# Autodesk Inventor assembly: Motorkühlung
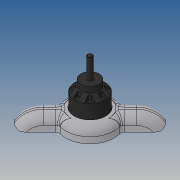
[picture p0: Inventor's stored thumbnail of the model, 180x180]
Saved by Autodesk Inventor 2019.4 (Build 234330000, 330)
## iProperties
Part Number: Motorkühlung
Document SubType Name: Assembly
Designer: Admin
Mass: 135.524 g
Surface Area: 242.561 cm^2
Volume: 41.9038 cm^3
Density: 3.23417 g/cm^3
Author: Admin
Revision: -
VAULT_Status: in Bearbeitung
Gewicht: 0,136 kg
InventorVersion: 2019.4
## Documents named in this file (4)
- C:\Users\tonn\Documents\GitHub\CAD_Elements\CAD\Hektor\Motorkühlung.iam
- Norm.iam
- C:\Users\tonn\Documents\GitHub\CAD_Elements\CAD\Motor\CobraCP2814-1050kv.ipt
- C:\Users\tonn\Documents\GitHub\CAD_Elements\CAD\Hektor\Motorkühlung.ipt
## Components (2 placed, 2 different names)
1. COBRACP2814-1050KV_COBRACP2814-1050KV--IPT:1 — Fluchtend:2, Passend:2, Passend:3
2. MOTORKÜHLUNG_MOTORKÜHLUNG--IPT:1 — Fluchtend:2, Passend:2, Passend:3
## Relationships (3: Mate 2, Flush 1)
- Fluchtend:2 [Flush]: COBRACP2814-1050KV_COBRACP2814-1050KV--IPT:1 ↔ MOTORKÜHLUNG_MOTORKÜHLUNG--IPT:1
- Passend:2 [Mate]: COBRACP2814-1050KV_COBRACP2814-1050KV--IPT:1 ↔ MOTORKÜHLUNG_MOTORKÜHLUNG--IPT:1
- Passend:3 [Mate]: COBRACP2814-1050KV_COBRACP2814-1050KV--IPT:1 ↔ MOTORKÜHLUNG_MOTORKÜHLUNG--IPT:1
## Named parameters: Gewicht = 0.135524
note: some values were not read from the file. Shown as the stored number, unit unknown: "Gewicht".
